# Autodesk Inventor assembly: CO-0-01-controlsBox
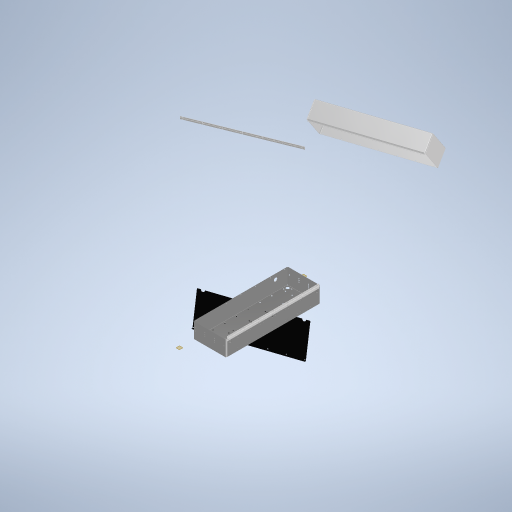
[picture p0: Inventor's stored thumbnail of the model, 512x512]
Saved by Autodesk Inventor 2023 (Build 270158000, 158)
## iProperties
Created: 2023-04-11
Part Number: CO-0-01-controlsBox
Document SubType Name: Weldment
Designer: t205b
Weld Material: Welded Aluminum-6061
Mass: 4095.48 g
Surface Area: 13841.4 cm^2
Volume: 1516.85 cm^3
Density: 2.7 g/cm^3
Author: t205b
## Documents named in this file (5)
- C:\Users\t205b\OneDrive\Documents\Github\BehrendURCMechanical\CAD\Controls\CO-0-04-controlsBoxProtocase.iam
- C:\Users\t205b\OneDrive\Documents\Github\BehrendURCMechanical\CAD\Controls\CO-1-04-controlsBox.ipt
- C:\Users\t205b\OneDrive\Documents\Github\BehrendURCMechanical\CAD\Controls\CO-1-02-controlsSeperator.ipt
- C:\Users\t205b\OneDrive\Documents\Github\BehrendURCMechanical\CAD\Controls\CO-1-02-controlsLid.ipt
- C:\Users\t205b\OneDrive\Documents\Github\BehrendURCMechanical\CAD\Controls\Tight-Clearance_Piano_Hinge.ipt
## Components (5 placed, 4 different names)
1. CO-1-04-controlsBox:1 — Mate:3, Mate:4, Mate:5, Mate:6
2. CO-1-02-controlsSeperator:1
3. CO-1-02-controlsLid:1
4. Tight-Clearance_Piano_Hinge:1
5. Tight-Clearance_Piano_Hinge:2 — Mate:5, Mate:6
## Relationships (5: Mate 5)
- [Mate]: CO-1-04-controlsBox:1
- Mate:3: CO-1-04-controlsBox:1
- Mate:4: CO-1-04-controlsBox:1
- Mate:5: CO-1-04-controlsBox:1 ↔ Tight-Clearance_Piano_Hinge:2
- Mate:6 (-10 mm): CO-1-04-controlsBox:1 ↔ Tight-Clearance_Piano_Hinge:2
